# Autodesk Inventor assembly: CDBEM
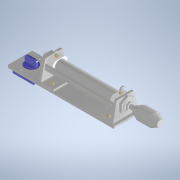
[picture p0: Inventor's stored thumbnail of the model, 180x180]
Saved by Autodesk Inventor 2022 (Build 260153000, 153)
## iProperties
Created: 2019-07-28
Part Number: CDBEM
Document SubType Name: Assembly
Designer: jmate
Sending System: Solid Edge
SolidEdgeDocType: Assembly
Template: Normal.asm
Last Saved Time: 2019-07-29
Densidad del cordón de soldadura: 0,000 g/cm^3
Author: jmate
Last Saved By: jmate
## Documents named in this file (14)
- C:\Users\jmate\Downloads\Stufy Stuff\JMT\S2\Computer-Aided Design\Segundo corte\Pistón Neumático\CDBEM.iam
- C:\Users\jmate\Downloads\Stufy Stuff\JMT\S2\Computer-Aided Design\Segundo corte\Pistón Neumático\PB.ipt
- C:\Users\jmate\Downloads\Stufy Stuff\JMT\S2\Computer-Aided Design\Segundo corte\Pistón Neumático\LL.ipt
- C:\Users\jmate\Downloads\Stufy Stuff\JMT\S2\Computer-Aided Design\Segundo corte\Pistón Neumático\PLPB.ipt
- C:\Users\jmate\Downloads\Stufy Stuff\JMT\S2\Computer-Aided Design\Segundo corte\Pistón Neumático\CL.ipt
- C:\Users\jmate\Downloads\Stufy Stuff\JMT\S2\Computer-Aided Design\Segundo corte\Pistón Neumático\EA.ipt
- C:\Users\jmate\Downloads\Stufy Stuff\JMT\S2\Computer-Aided Design\Segundo corte\Pistón Neumático\TR1.ipt
- C:\Users\jmate\Downloads\Stufy Stuff\JMT\S2\Computer-Aided Design\Segundo corte\Pistón Neumático\PT.ipt
- C:\Users\jmate\Downloads\Stufy Stuff\JMT\S2\Computer-Aided Design\Segundo corte\Pistón Neumático\TR2.ipt
- C:\Users\jmate\Downloads\Stufy Stuff\JMT\S2\Computer-Aided Design\Segundo corte\Pistón Neumático\RM.ipt
- C:\Users\jmate\Downloads\Stufy Stuff\JMT\S2\Computer-Aided Design\Segundo corte\Pistón Neumático\3MM.ipt
- C:\Users\jmate\Downloads\Stufy Stuff\JMT\S2\Computer-Aided Design\Segundo corte\Pistón Neumático\AG1.ipt
- C:\Users\jmate\Downloads\Stufy Stuff\JMT\S2\Computer-Aided Design\Segundo corte\Pistón Neumático\AG2.ipt
- C:\Users\jmate\Downloads\Stufy Stuff\JMT\S2\Computer-Aided Design\Segundo corte\Pistón Neumático\LGR.ipt
## Components (24 placed, 13 different names)
1. PB.par:1 — Coincidencia:11, Coincidencia:12, Nivelación:1, Nivelación:2, Coincidencia:16, Coincidencia:19, Coincidencia:20, Coincidencia:21, Coincidencia:27, Coincidencia:28, Coincidencia:29, Coincidencia:30, Coincidencia:34, Nivelación:3, Coincidencia:35, Coincidencia:36, Coincidencia:37, Coincidencia:38, Coincidencia:39
2. LL.psm:1 — Coincidencia:6, Coincidencia:7, Coincidencia:8, Coincidencia:11, Coincidencia:12, Coincidencia:13, Coincidencia:14, Coincidencia:15, Nivelación:1, Coincidencia:42
3. LL.psm:2 — Nivelación:2, Coincidencia:16, Coincidencia:17, Coincidencia:18, Coincidencia:19, Coincidencia:26, Coincidencia:31, Ángulo:1, Nivelación:4
4. PLPB.par:1 — Coincidencia:34, Nivelación:3, Coincidencia:35
5. CL.par:1 — Coincidencia:1, Coincidencia:2, Coincidencia:3, Coincidencia:4, Coincidencia:5, Coincidencia:6, Coincidencia:7, Coincidencia:9, Coincidencia:10, Coincidencia:32, Coincidencia:33, Ángulo:1, Nivelación:4, Coincidencia:40, Coincidencia:41, Coincidencia:43, Coincidencia:44
6. EA.par:1 — Coincidencia:3, Coincidencia:9
7. EA.par:2 — Coincidencia:4, Coincidencia:10
8. TR1.par:1 — Coincidencia:26, Coincidencia:31
9. TR1.par:2 — Coincidencia:5, Coincidencia:8
10. PT.par:1 — Coincidencia:1, Coincidencia:2
11. TR2.par:1 — Coincidencia:32, Coincidencia:33
12. RM.par:1 — Coincidencia:17
13. RM.par:2 — Coincidencia:18
14. RM.par:3 — Coincidencia:13, Coincidencia:14
15. RM.par:4 — Coincidencia:15
16. 3MM.par:1 — Coincidencia:38, Coincidencia:39
17. 3MM.par:2 — Coincidencia:36, Coincidencia:37
18. AG1.par:1 — Coincidencia:28, Coincidencia:29
19. 3MM.par:3 — Coincidencia:20
20. AG2.par:1 — Coincidencia:27, Coincidencia:30
21. 3MM.par:4 — Coincidencia:21
22. LGR.par:1 — Coincidencia:42, Coincidencia:43, Coincidencia:44
23. 3MM.par:5 — Coincidencia:40
24. 3MM.par:6 — Coincidencia:41
## Relationships (45: Mate 40, Flush 4, Angle 1)
- Coincidencia:1 [Mate]: CL.par:1 ↔ PT.par:1
- Coincidencia:2 [Mate]: CL.par:1 ↔ PT.par:1
- Coincidencia:3 [Mate]: CL.par:1 ↔ EA.par:1
- Coincidencia:4 [Mate]: CL.par:1 ↔ EA.par:2
- Coincidencia:5 [Mate]: CL.par:1 ↔ TR1.par:2
- Coincidencia:6 [Mate]: LL.psm:1 ↔ CL.par:1
- Coincidencia:7 [Mate]: LL.psm:1 ↔ CL.par:1
- Coincidencia:8 [Mate]: LL.psm:1 ↔ TR1.par:2
- Coincidencia:9 [Mate]: CL.par:1 ↔ EA.par:1
- Coincidencia:10 [Mate]: CL.par:1 ↔ EA.par:2
- Coincidencia:11 [Mate]: PB.par:1 ↔ LL.psm:1
- Coincidencia:12 [Mate]: PB.par:1 ↔ LL.psm:1
- Coincidencia:13 [Mate]: LL.psm:1 ↔ RM.par:3
- Coincidencia:14 [Mate]: LL.psm:1 ↔ RM.par:3
- Coincidencia:15 [Mate]: LL.psm:1 ↔ RM.par:4
- Nivelación:1 [Flush]: PB.par:1 ↔ LL.psm:1
- Nivelación:2 [Flush]: PB.par:1 ↔ LL.psm:2
- Coincidencia:16 [Mate]: PB.par:1 ↔ LL.psm:2
- Coincidencia:17 [Mate]: LL.psm:2 ↔ RM.par:1
- Coincidencia:18 [Mate]: LL.psm:2 ↔ RM.par:2
- Coincidencia:19 [Mate]: PB.par:1 ↔ LL.psm:2
- Coincidencia:20 [Mate]: PB.par:1 ↔ 3MM.par:3
- Coincidencia:21 [Mate]: PB.par:1 ↔ 3MM.par:4
- Coincidencia:26 [Mate]: LL.psm:2 ↔ TR1.par:1
- Coincidencia:27 [Mate]: PB.par:1 ↔ AG2.par:1
- Coincidencia:28 [Mate]: PB.par:1 ↔ AG1.par:1
- Coincidencia:29 [Mate]: PB.par:1 ↔ AG1.par:1
- Coincidencia:30 [Mate]: PB.par:1 ↔ AG2.par:1
- Coincidencia:31 [Mate]: LL.psm:2 ↔ TR1.par:1
- Coincidencia:32 [Mate]: CL.par:1 ↔ TR2.par:1
- Coincidencia:33 [Mate]: CL.par:1 ↔ TR2.par:1
- Coincidencia:34 [Mate]: PB.par:1 ↔ PLPB.par:1
- Nivelación:3 [Flush]: PB.par:1 ↔ PLPB.par:1
- Coincidencia:35 [Mate]: PB.par:1 ↔ PLPB.par:1
- Coincidencia:36 [Mate]: PB.par:1 ↔ 3MM.par:2
- Coincidencia:37 [Mate]: PB.par:1 ↔ 3MM.par:2
- Coincidencia:38 [Mate]: PB.par:1 ↔ 3MM.par:1
- Coincidencia:39 [Mate]: PB.par:1 ↔ 3MM.par:1
- Ángulo:1 [Angle] (90 deg): LL.psm:2 ↔ CL.par:1
- Nivelación:4 [Flush] (-2.643 mm): LL.psm:2 ↔ CL.par:1
- Coincidencia:40 [Mate]: CL.par:1 ↔ 3MM.par:5
- Coincidencia:41 [Mate]: CL.par:1 ↔ 3MM.par:6
- Coincidencia:42 [Mate]: LL.psm:1 ↔ LGR.par:1
- Coincidencia:43 [Mate]: CL.par:1 ↔ LGR.par:1
- Coincidencia:44 [Mate]: CL.par:1 ↔ LGR.par:1
